# Autodesk Inventor assembly: 3D_skenner
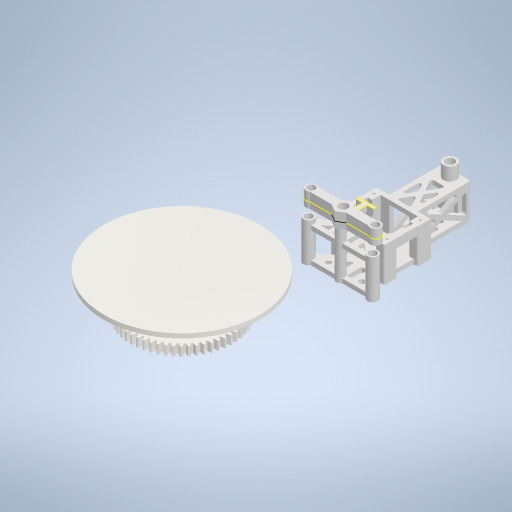
[picture p0: Inventor's stored thumbnail of the model, 512x512]
Saved by Autodesk Inventor 2023 (Build 270158000, 158)
## iProperties
Created: 2022-09-12
Part Number: 3D_skenner
Document SubType Name: Assembly
Designer: simon
Author: simon
## Documents named in this file (12)
- C:\Users\simon\OneDrive\Namizje\school\4. letnik\Matura\Izdelek\Izdelovanje\3D model\3D_skenner.iam
- C:\Users\simon\OneDrive\Namizje\school\4. letnik\Matura\Izdelek\Izdelovanje\3D model\Ogrodje_spodaj_1.ipt
- C:\Users\simon\OneDrive\Namizje\school\4. letnik\Matura\Izdelek\Izdelovanje\3D model\motor_sample.ipt
- C:\Users\simon\OneDrive\Namizje\school\4. letnik\Matura\Izdelek\Izdelovanje\3D model\motorni_zobnik.ipt
- C:\Users\simon\OneDrive\Namizje\school\4. letnik\Matura\Izdelek\Izdelovanje\3D model\Zobnik_na plošči.ipt
- C:\Users\simon\OneDrive\Namizje\school\4. letnik\Matura\Izdelek\Izdelovanje\3D model\3D_skenner\Design Accelerator\Spur Gears1.iam
- C:\Users\simon\OneDrive\Namizje\school\4. letnik\Matura\Izdelek\Izdelovanje\3D model\3D_skenner\Design Accelerator\Drzalo_motorja.ipt
- C:\Users\simon\OneDrive\Namizje\school\4. letnik\Matura\Izdelek\Izdelovanje\3D model\3D_skenner\Design Accelerator\Spur Gears1_CPY.iam
- C:\Users\simon\OneDrive\Namizje\school\4. letnik\Matura\Izdelek\Izdelovanje\3D model\združevalnik_osi.ipt
- C:\Users\simon\OneDrive\Namizje\school\4. letnik\Matura\Izdelek\Izdelovanje\3D model\¸držalo_laserja.ipt
- C:\Users\simon\OneDrive\Namizje\school\4. letnik\Matura\Izdelek\Izdelovanje\3D model\test_izbrisi.ipt
- C:\Users\simon\OneDrive\Namizje\school\4. letnik\Matura\Izdelek\Izdelovanje\3D model\chep_za_os.ipt
## Components (11 placed, 11 different names)
1. Ogrodje_spodaj_1:1 — Flush:1, Flush:3
2. motor_sample:1 — Rigid:1
3. motorni_zobnik:1
4. Zobnik_na plošči:1
5. Spur Gears:1 [sub-assembly] — Rigid:1
6. Drzalo_motorja:1 — Flush:1
7. Spur Gears1_CPY:1 [sub-assembly] — Flush:2
8. združevalnik_osi:1 — Flush:2
9. ¸držalo_laserja:1 — Flush:3, Flush:4, Flush:5
10. test_izbrisi:1 — Flush:4
11. chep_za_os:1 — Flush:5
## Relationships (6: Flush 5, WeldJoint 1)
- Rigid:1 [WeldJoint]: motor_sample:1 ↔ Spur Gears:1
- Flush:1: Ogrodje_spodaj_1:1 ↔ Drzalo_motorja:1
- Flush:2: Spur Gears1_CPY:1 ↔ združevalnik_osi:1
- Flush:3: Ogrodje_spodaj_1:1 ↔ ¸držalo_laserja:1
- Flush:4: ¸držalo_laserja:1 ↔ test_izbrisi:1
- Flush:5: ¸držalo_laserja:1 ↔ chep_za_os:1
